# Autodesk Inventor assembly: 3PinBlock
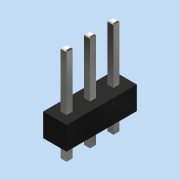
[picture p0: Inventor's stored thumbnail of the model, 180x180]
Saved by Autodesk Inventor 2017 (Build 210142000, 142)
## iProperties
Created: 2017-01-25
Part Number: 3PinBlock
Document SubType Name: Assembly
Designer: techn
Author: techn
## Documents named in this file (2)
- D:\OneDrive\Documents\Other Projects\Submarine\CAD\midships\ElectronicsSection\ServoController\3PinBlock.iam
- D:\OneDrive\Documents\Other Projects\Submarine\CAD\midships\ElectronicsSection\ServoController\PinBlock.iam
## Components (3 placed, 1 different names)
1. PinBlock:1 [sub-assembly] — Flush:3, Flush:4, Mate:2
2. PinBlock:2 [sub-assembly] — Mate:1, Flush:1, Flush:2, Flush:3, Flush:4, Mate:2
3. PinBlock:3 [sub-assembly] — Mate:1, Flush:1, Flush:2
## Relationships (6: Flush 4, Mate 2)
- Mate:1: PinBlock:2 ↔ PinBlock:3
- Flush:1: PinBlock:2 ↔ PinBlock:3
- Flush:2: PinBlock:2 ↔ PinBlock:3
- Flush:3: PinBlock:1 ↔ PinBlock:2
- Flush:4: PinBlock:1 ↔ PinBlock:2
- Mate:2: PinBlock:1 ↔ PinBlock:2
